# Autodesk Inventor assembly: Arm8
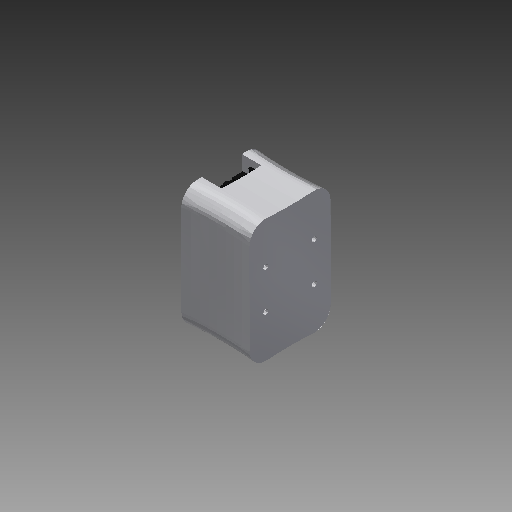
[picture p0: Inventor's stored thumbnail of the model, 512x512]
Saved by Autodesk Inventor 2017 SP1 (Build 210196100, 196)
## iProperties
Created: 2018-03-03
Part Number: Arm8
Document SubType Name: Assembly
Designer: Zach
Author: Zach
## Documents named in this file (2)
- C:\Users\Zach\Documents\GitHub\tr1_description\meshes\Visual Assembly\Arm8.iam
- C:\Users\Zach\Desktop\Arm8.ipt
## Components (1 placed, 1 different names)
1. Arm8:1 — Mate:1, Mate:2, Mate:3
## Relationships (3: Mate 3)
- Mate:1: Arm8:1
- Mate:2: Arm8:1
- Mate:3: Arm8:1
